# Autodesk Inventor assembly: Assembly1
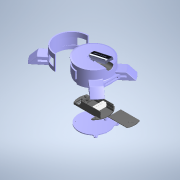
[picture p0: Inventor's stored thumbnail of the model, 180x180]
Saved by Autodesk Inventor 2020 (Build 240168000, 168)
## iProperties
Created: 2020-11-24
Part Number: Assembly1
Document SubType Name: Assembly
Designer: sandr
Author: sandr
## Documents named in this file (11)
- C:\Users\sandr\OneDrive\Formacion\Universidad\2020-2\Fundamentos de biodiseño\Modelado\Case v3\assembly explotado.iam
- C:\Users\sandr\OneDrive\Formacion\Universidad\2020-2\Fundamentos de biodiseño\Modelado\Case v3\Core.ipt
- C:\Users\sandr\OneDrive\Formacion\Universidad\2020-2\Fundamentos de biodiseño\Modelado\Case v3\coupling_core.ipt
- C:\Users\sandr\OneDrive\Formacion\Universidad\2020-2\Fundamentos de biodiseño\Modelado\Case v3\case_frec_res.ipt
- C:\Users\sandr\OneDrive\Formacion\Universidad\2020-2\Fundamentos de biodiseño\Modelado\Case v3\cover_battery.ipt
- C:\Users\sandr\OneDrive\Formacion\Universidad\2020-2\Fundamentos de biodiseño\Modelado\Case v3\cover_case_frec_res.ipt
- C:\Users\sandr\OneDrive\Formacion\Universidad\2020-2\Fundamentos de biodiseño\Modelado\Case v3\cover_core.ipt
- C:\Users\sandr\OneDrive\Formacion\Universidad\2020-2\Fundamentos de biodiseño\Modelado\Case v3\PPG_cover.ipt
- C:\Users\sandr\OneDrive\Formacion\Universidad\2020-2\Fundamentos de biodiseño\Modelado\Case v3\reflec_frec_res.ipt
- C:\Users\sandr\OneDrive\Formacion\Universidad\2020-2\Fundamentos de biodiseño\Modelado\Case v3\fastener ppg.ipt
- C:\Users\sandr\OneDrive\Formacion\Universidad\2020-2\Fundamentos de biodiseño\Modelado\Case v3\battery_contact.ipt
## Components (10 placed, 10 different names)
1. Core:1 — Insert:1, Insert:2, Mate:1, Mate:2, Mate:3, Flush:1, Flush:2, Flush:3, Mate:5, Mate:6, Mate:10, Mate:11
2. coupling_core:1 — Flush:1, Flush:2
3. case_frec_res:1 — Slider:1, Slider:2, Mate:8, Mate:9
4. cover_battery:1 — Mate:13, Mate:14
5. cover_case_frec_res:1 — Slider:2
6. cover_core:1 — Mate:10, Mate:11, Mate:13, Mate:14
7. PPG_cover:1 — Insert:1
8. reflec_frec_res:1 — Slider:1
9. fastener ppg:1 — Insert:2
10. battery_contact:1 — Mate:1, Mate:2, Mate:3
## Relationships (18: Mate 11, Flush 3, TranslationJoint 2, Insert 2)
- Slider:1 [TranslationJoint] (0.2 mm): case_frec_res:1 ↔ reflec_frec_res:1
- Slider:2 [TranslationJoint]: case_frec_res:1 ↔ cover_case_frec_res:1
- Insert:1: Core:1 ↔ PPG_cover:1
- Insert:2: Core:1 ↔ fastener ppg:1
- Mate:1: Core:1 ↔ battery_contact:1
- Mate:2: Core:1 ↔ battery_contact:1
- Mate:3: Core:1 ↔ battery_contact:1
- Flush:1: Core:1 ↔ coupling_core:1
- Flush:2: Core:1 ↔ coupling_core:1
- Flush:3: Core:1
- Mate:5: Core:1
- Mate:6: Core:1
- Mate:8: case_frec_res:1
- Mate:9: case_frec_res:1
- Mate:10: Core:1 ↔ cover_core:1
- Mate:11: Core:1 ↔ cover_core:1
- Mate:13: cover_battery:1 ↔ cover_core:1
- Mate:14: cover_battery:1 ↔ cover_core:1
